# Autodesk Inventor assembly: Assembly1
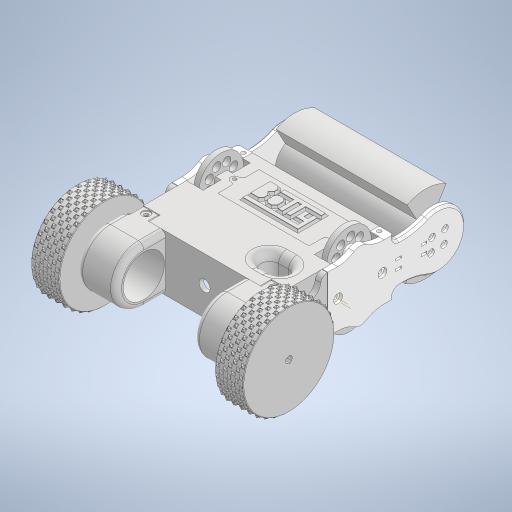
[picture p0: Inventor's stored thumbnail of the model, 512x512]
Saved by Autodesk Inventor 2024.2 (Build 282272000, 272)
## iProperties
Created: 2024-03-13
Part Number: Assembly1
Document SubType Name: Assembly
Designer: jerem
Author: jerem
## Documents named in this file (10)
- C:\Users\jerem\OneDrive\WRCL Botty\CAD\Assembly1.iam
- C:\Users\jerem\OneDrive\WRCL Botty\CAD\Cover.ipt
- C:\Users\jerem\OneDrive\WRCL Botty\CAD\NEW_BODY.ipt
- C:\Users\jerem\OneDrive\WRCL Botty\CAD\small_wheel.ipt
- C:\Users\jerem\OneDrive\WRCL Botty\CAD\wheel_bracket_new.ipt
- C:\Users\jerem\OneDrive\WRCL Botty\CAD\bldc_arm.ipt
- C:\Users\jerem\OneDrive\WRCL Botty\CAD\bearing_arm.ipt
- C:\Users\jerem\OneDrive\WRCL Botty\CAD\newDrum.ipt
- C:\Users\jerem\OneDrive\WRCL Botty\CAD\big_wheel.ipt
- C:\Users\jerem\OneDrive\WRCL Botty\CAD\Battery_Cover.ipt
## Components (14 placed, 9 different names)
1. Cover:1 — Mate:1, Mate:2, Mate:5
2. NEW_BODY:1 — Mate:1, Mate:2, Mate:5, Mate:16, Mate:25, Mate:26, Mate:27, Mate:29, Mate:30, Mate:31, Mate:38, Mate:39, Mate:40, Mate:41, Mate:42, Mate:43, Mate:44, Mate:51, Mate:52, Mate:54, Mate:55, Mate:56, Mate:57, Mate:58
3. small_wheel:1 — Mate:32, Mate:34
4. small_wheel:2 — Mate:33, Mate:35
5. small_wheel:3 — Mate:38, Mate:39
6. small_wheel:4 — Mate:40, Mate:41
7. wheel_bracket_new:1 — Mate:26, Mate:49, Mate:50, Mate:51, Mate:52
8. wheel_bracket_new:2 — Mate:16, Mate:48, Mate:53, Mate:54, Mate:55
9. bldc_arm:1 — Mate:29, Mate:30, Mate:31, Mate:32, Mate:33, Mate:34, Mate:35, Mate:45
10. bearing_arm:1 — Mate:42, Mate:43, Mate:44, Mate:46
11. newDrum:1 — Mate:45, Mate:46
12. big_wheel:1 — Mate:48, Mate:53
13. big_wheel:2 — Mate:49, Mate:50
14. Battery_Cover:1 — Mate:56, Mate:57, Mate:58
## Relationships (34: Mate 34)
- Mate:1: Cover:1 ↔ NEW_BODY:1
- Mate:2: Cover:1 ↔ NEW_BODY:1
- Mate:5: Cover:1 ↔ NEW_BODY:1
- Mate:16: NEW_BODY:1 ↔ wheel_bracket_new:2
- Mate:25: NEW_BODY:1
- Mate:26: NEW_BODY:1 ↔ wheel_bracket_new:1
- Mate:27: NEW_BODY:1
- Mate:29: NEW_BODY:1 ↔ bldc_arm:1
- Mate:30: NEW_BODY:1 ↔ bldc_arm:1
- Mate:31: NEW_BODY:1 ↔ bldc_arm:1
- Mate:32: small_wheel:1 ↔ bldc_arm:1
- Mate:33: small_wheel:2 ↔ bldc_arm:1
- Mate:34: small_wheel:1 ↔ bldc_arm:1
- Mate:35: small_wheel:2 ↔ bldc_arm:1
- Mate:38: NEW_BODY:1 ↔ small_wheel:3
- Mate:39: NEW_BODY:1 ↔ small_wheel:3
- Mate:40: NEW_BODY:1 ↔ small_wheel:4
- Mate:41: NEW_BODY:1 ↔ small_wheel:4
- Mate:42: NEW_BODY:1 ↔ bearing_arm:1
- Mate:43: NEW_BODY:1 ↔ bearing_arm:1
- Mate:44: NEW_BODY:1 ↔ bearing_arm:1
- Mate:45: bldc_arm:1 ↔ newDrum:1
- Mate:46: bearing_arm:1 ↔ newDrum:1
- Mate:48: wheel_bracket_new:2 ↔ big_wheel:1
- Mate:49: wheel_bracket_new:1 ↔ big_wheel:2
- Mate:50: wheel_bracket_new:1 ↔ big_wheel:2
- Mate:51: NEW_BODY:1 ↔ wheel_bracket_new:1
- Mate:52: NEW_BODY:1 ↔ wheel_bracket_new:1
- Mate:53: wheel_bracket_new:2 ↔ big_wheel:1
- Mate:54: NEW_BODY:1 ↔ wheel_bracket_new:2
- Mate:55: NEW_BODY:1 ↔ wheel_bracket_new:2
- Mate:56: NEW_BODY:1 ↔ Battery_Cover:1
- Mate:57: NEW_BODY:1 ↔ Battery_Cover:1
- Mate:58: NEW_BODY:1 ↔ Battery_Cover:1
